# Autodesk Inventor assembly: Arm 2.0 Assembly
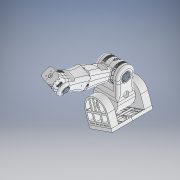
[picture p0: Inventor's stored thumbnail of the model, 180x180]
Saved by Autodesk Inventor 2017 SP1 (Build 210196100, 196)
## iProperties
Created: 2017-09-28
Part Number: Arm 2.0 Assembly
Document SubType Name: Assembly
Designer: Zach
Author: Zach
## Documents named in this file (20)
- C:\Users\Zach\Documents\GitHub\tr1\src\Body\Arm 2.0 Assembly\Arm 2.0 Assembly.iam
- C:\Users\Zach\Documents\GitHub\tr1\src\Body\Arm 2.0 Assembly\AA001.ipt
- C:\Users\Zach\Documents\GitHub\tr1\src\Body\Arm 2.0 Assembly\Steel Rod 8mm x 135mm.ipt
- C:\Users\Zach\Documents\GitHub\tr1\lib\22x8x8mm Bearing.ipt
- C:\Users\Zach\Documents\GitHub\tr1\src\Body\Arm 2.0 Assembly\AA002.ipt
- C:\Users\Zach\Documents\GitHub\tr1\src\Body\Arm 2.0 Assembly\AA003.ipt
- C:\Users\Zach\Documents\GitHub\tr1\src\Body\Arm 2.0 Assembly\AA004.ipt
- C:\Users\Zach\Documents\GitHub\tr1\src\Body\Arm 2.0 Assembly\AA005.ipt
- C:\Users\Zach\Documents\GitHub\tr1\src\Body\Arm 2.0 Assembly\AA006.ipt
- C:\Users\Zach\Documents\GitHub\tr1\src\Body\Arm 2.0 Assembly\AA007.ipt
- C:\Users\Zach\Documents\GitHub\tr1\lib\QS12MM250\QS12MM250.ipt
- C:\Users\Zach\Documents\GitHub\tr1\src\Body\Arm 2.0 Assembly\AA008.ipt
- C:\Users\Zach\Documents\GitHub\tr1\src\Body\Arm 2.0 Assembly\AA009.ipt
- C:\Users\Zach\Documents\GitHub\tr1\lib\13x4x5mm Bearing.ipt
- C:\Users\Zach\Documents\GitHub\tr1\src\Body\Arm 2.0 Assembly\AA010.ipt
- C:\Users\Zach\Documents\GitHub\tr1\src\Body\Arm 2.0 Assembly\AA011.ipt
- C:\Users\Zach\Documents\GitHub\tr1\src\Body\Arm 2.0 Assembly\AA012.ipt
- C:\Users\Zach\Documents\GitHub\tr1\src\Body\Arm 2.0 Assembly\Steel Rod 8mm x 100mm.ipt
- C:\Users\Zach\Documents\GitHub\tr1\src\Body\Arm 2.0 Assembly\AA013.ipt
- C:\Users\Zach\Documents\GitHub\tr1\src\Body\Arm 2.0 Assembly\AA014.ipt
## Components (31 placed, 19 different names)
1. AA001:1 — Mate:1, Mate:3, Flush:1, Mate:4, Flush:2, Mate:7, Mate:9, Mate:10, Mate:11, Mate:58, Mate:59, Mate:60, Mate:61, Mate:62, Mate:63
2. AA002:2 — Flush:4, Mate:5, Mate:8, Mate:14, Mate:28, Mate:29, Mate:34
3. AA003:1 — Flush:4, Mate:5, Mate:6, Mate:7, Mate:8, Mate:27, Mate:32
4. AA004:1 — Mate:9, Mate:10, Mate:11, Mate:12, Mate:13, Mate:15, Mate:23, Mate:26
5. AA005:1 — Mate:16, Mate:17, Mate:18, Mate:26
6. AA006:1 — Mate:21, Mate:22, Mate:24, Mate:25
7. AA007:1 — Mate:16, Mate:17, Mate:18, Mate:19, Mate:20
8. AA007:2 — Mate:19, Mate:20, Mate:21, Mate:22
9. AA008:1 — Mate:27, Mate:28, Mate:29, Mate:30, Mate:31, Mate:33, Mate:35, Mate:36, Mate:39, Mate:41, Mate:43, Mate:46, Mate:47
10. AA009:1 — Mate:30, Mate:31
11. AA008:2 — Mate:32, Mate:33, Mate:34, Mate:37, Mate:38, Mate:40, Mate:42, Mate:44, Mate:45, Mate:48
12. AA010:1 — Mate:47, Mate:48, Mate:52, Mate:53, Mate:55, Flush:6, Mate:56, Flush:7, Flush:8, Mate:64, Mate:65, Mate:66, Mate:67, Mate:68, Mate:69
13. AA011:1 — Mate:49, Mate:50, Mate:51
14. AA012:1 — Mate:49, Mate:50, Mate:51, Mate:52, Mate:53
15. AA013:1 — Mate:58, Mate:59, Mate:60
16. AA013:2 — Mate:61, Mate:62, Mate:63
17. AA014:1 — Mate:64, Mate:65, Mate:66
18. AA014:2 — Mate:67, Mate:68, Mate:69
19. 13x4x5mm Bearing:1 — Mate:35, Mate:36
20. 13x4x5mm Bearing:2 — Mate:37, Mate:38
21. 13x4x5mm Bearing:3 — Mate:40, Mate:44
22. 13x4x5mm Bearing:4 — Mate:39, Mate:43
23. 13x4x5mm Bearing:5 — Mate:42, Mate:45
24. 13x4x5mm Bearing:6 — Mate:41, Mate:46
25. 22x8x8mm Bearing:1 — Mate:3, Flush:1, Flush:3
26. 22x8x8mm Bearing:2 — Mate:4, Flush:2
27. 22x8x8mm Bearing:3 — Mate:55, Flush:6, Mate:57
28. 22x8x8mm Bearing:4 — Mate:56, Flush:7
29. QS12MM250:1 — Mate:23, Mate:24, Mate:25
30. Steel Rod 8mm x 135mm:1 — Mate:1, Flush:3, Mate:6
31. Steel Rod 8mm x 100mm:1 — Mate:57, Flush:8
## Relationships (74: Mate 67, Flush 7)
- Mate:1: AA001:1 ↔ Steel Rod 8mm x 135mm:1
- Mate:3: AA001:1 ↔ 22x8x8mm Bearing:1
- Flush:1: AA001:1 ↔ 22x8x8mm Bearing:1
- Mate:4: AA001:1 ↔ 22x8x8mm Bearing:2
- Flush:2: AA001:1 ↔ 22x8x8mm Bearing:2
- Flush:3 (-2.5 mm): 22x8x8mm Bearing:1 ↔ Steel Rod 8mm x 135mm:1
- Flush:4: AA002:2 ↔ AA003:1
- Mate:5: AA002:2 ↔ AA003:1
- Mate:6: AA003:1 ↔ Steel Rod 8mm x 135mm:1
- Mate:7 (0.75 mm): AA001:1 ↔ AA003:1
- Mate:8: AA002:2 ↔ AA003:1
- Mate:9: AA001:1 ↔ AA004:1
- Mate:10: AA001:1 ↔ AA004:1
- Mate:11: AA001:1 ↔ AA004:1
- Mate:12: AA004:1
- Mate:13: AA004:1
- Mate:14: AA002:2
- Mate:15: AA004:1
- Mate:16: AA005:1 ↔ AA007:1
- Mate:17: AA005:1 ↔ AA007:1
- Mate:18: AA005:1 ↔ AA007:1
- Mate:19: AA007:1 ↔ AA007:2
- Mate:20: AA007:1 ↔ AA007:2
- Mate:21: AA006:1 ↔ AA007:2
- Mate:22: AA006:1 ↔ AA007:2
- Mate:23: AA004:1 ↔ QS12MM250:1
- Mate:24: AA006:1 ↔ QS12MM250:1
- Mate:25: AA006:1 ↔ QS12MM250:1
- Mate:26 (30 mm): AA004:1 ↔ AA005:1
- Mate:27: AA003:1 ↔ AA008:1
- Mate:28: AA002:2 ↔ AA008:1
- Mate:29: AA002:2 ↔ AA008:1
- Mate:30: AA008:1 ↔ AA009:1
- Mate:31: AA008:1 ↔ AA009:1
- Mate:32: AA003:1 ↔ AA008:2
- Mate:33: AA008:1 ↔ AA008:2
- Mate:34: AA002:2 ↔ AA008:2
- Mate:35: AA008:1 ↔ 13x4x5mm Bearing:1
- Mate:36: AA008:1 ↔ 13x4x5mm Bearing:1
- Mate:37: AA008:2 ↔ 13x4x5mm Bearing:2
- Mate:38: AA008:2 ↔ 13x4x5mm Bearing:2
- Mate:39: AA008:1 ↔ 13x4x5mm Bearing:4
- Mate:40: AA008:2 ↔ 13x4x5mm Bearing:3
- Mate:41: AA008:1 ↔ 13x4x5mm Bearing:6
- Mate:42: AA008:2 ↔ 13x4x5mm Bearing:5
- Mate:43: AA008:1 ↔ 13x4x5mm Bearing:4
- Mate:44: AA008:2 ↔ 13x4x5mm Bearing:3
- Mate:45: AA008:2 ↔ 13x4x5mm Bearing:5
- Mate:46: AA008:1 ↔ 13x4x5mm Bearing:6
- Mate:47: AA008:1 ↔ AA010:1
- Mate:48 (2.5 mm): AA008:2 ↔ AA010:1
- Mate:49: AA011:1 ↔ AA012:1
- Mate:50: AA011:1 ↔ AA012:1
- Mate:51: AA011:1 ↔ AA012:1
- Mate:52: AA010:1 ↔ AA012:1
- Mate:53 (1.75 mm): AA010:1 ↔ AA012:1
- Mate:55: AA010:1 ↔ 22x8x8mm Bearing:3
- Flush:6: AA010:1 ↔ 22x8x8mm Bearing:3
- Mate:56: AA010:1 ↔ 22x8x8mm Bearing:4
- Flush:7: AA010:1 ↔ 22x8x8mm Bearing:4
- Mate:57: 22x8x8mm Bearing:3 ↔ Steel Rod 8mm x 100mm:1
- Flush:8 (2.5 mm): AA010:1 ↔ Steel Rod 8mm x 100mm:1
- Mate:58: AA001:1 ↔ AA013:1
- Mate:59: AA001:1 ↔ AA013:1
- Mate:60: AA001:1 ↔ AA013:1
- Mate:61: AA001:1 ↔ AA013:2
- Mate:62: AA001:1 ↔ AA013:2
- Mate:63: AA001:1 ↔ AA013:2
- Mate:64: AA010:1 ↔ AA014:1
- Mate:65: AA010:1 ↔ AA014:1
- Mate:66: AA010:1 ↔ AA014:1
- Mate:67: AA010:1 ↔ AA014:2
- Mate:68: AA010:1 ↔ AA014:2
- Mate:69: AA010:1 ↔ AA014:2
